# Autodesk Inventor assembly: RCS
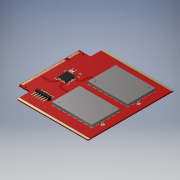
[picture p0: Inventor's stored thumbnail of the model, 180x180]
Saved by Autodesk Inventor 2018 (Build 220112000, 112)
## iProperties
Created: 2018-07-04
Part Number: RCS
Document SubType Name: Assembly
Designer: Bradley
Author: Bradley
## Documents named in this file (10)
- D:\Users\Bradley\Documents\CougsInSpace\CougSat1-Hardware\CougSat1-RadioBoard\CADModel\Native\Comms.iam
- D:\Users\Bradley\Documents\CougsInSpace\CougSat1-Hardware\CougSat1-RadioBoard\CADModel\Native\Comms_PCB.ipt
- D:\Users\Bradley\Documents\CougsInSpace\Resources\ComponentModels\Connectors\U.FL_Male.ipt
- D:\Users\Bradley\Documents\CougsInSpace\Resources\ComponentModels\Electronics\Crystal_ECX-42.ipt
- D:\Users\Bradley\Documents\CougsInSpace\Resources\ComponentModels\Electronics\LED_1608.ipt
- D:\Users\Bradley\Documents\CougsInSpace\Resources\ComponentModels\Connectors\SMD2.54-1x06-R.ipt
- D:\Users\Bradley\Documents\CougsInSpace\Resources\ComponentModels\Electronics\Shield_Frame-40x30mm.ipt
- D:\Users\Bradley\Documents\CougsInSpace\Resources\ComponentModels\Electronics\Shield_Cover-40x30mm.ipt
- D:\Users\Bradley\Documents\CougsInSpace\Resources\ComponentModels\Electronics\Capacitor_1608-0.8mm.ipt
- D:\Users\Bradley\Documents\CougsInSpace\Resources\ComponentModels\Electronics\Semiconductor_QFP64-10x10.ipt
## Components (17 placed, 9 different names)
1. Comms_PCB:1 — Mate:11, Mate:12, Mate:16, Mate:20, Flush:14, Mate:21, Mate:22, Flush:15, Mate:23, Flush:16, Flush:17, Mate:24, Flush:18, Flush:19, Mate:25, Mate:26, Mate:27, Mate:28, Mate:33, Flush:21, Flush:22, Mate:34, Mate:35, Mate:36, Mate:37, Flush:27, Mate:29, Mate:30, Mate:38, Mate:39, Flush:30, Flush:31, Mate:31, Mate:40, Flush:33, Mate:32, Mate:41, Flush:35
2. U.FL_Male:1 — Flush:11, Mate:2, Mate:11, Flush:12, Flush:13
3. Crystal_ECX-42:1 — Mate:24, Flush:18, Flush:19
4. LED_1608:1 — Mate:31, Mate:40, Flush:33
5. SMD2.54-1x06-R:1 — Mate:23, Flush:16, Flush:17
6. U.FL_Male:2 — Mate:12, Flush:12, Flush:13
7. Shield_Frame-40x30mm:1 — Mate:13, Mate:14, Mate:15, Mate:16, Flush:14, Mate:21
8. Shield_Cover-40x30mm:1 — Mate:13, Mate:14, Mate:15
9. Shield_Frame-40x30mm:2 — Mate:20, Mate:22, Flush:15
10. Shield_Cover-40x30mm:2
11. Capacitor_1608-0.8mm:1 — Mate:26, Flush:22, Mate:36
12. Capacitor_1608-0.8mm:2 — Mate:27, Flush:21, Mate:37
13. Capacitor_1608-0.8mm:3 — Mate:25, Mate:34, Mate:35
14. Capacitor_1608-0.8mm:4 — Mate:28, Mate:33, Flush:27
15. Capacitor_1608-0.8mm:5 — Mate:30, Mate:38, Flush:30
16. Capacitor_1608-0.8mm:6 — Mate:29, Mate:39, Flush:31
17. Semiconductor_QFP64-10x10:1 — Mate:32, Mate:41, Flush:35
## Relationships (48: Mate 32, Flush 16)
- Flush:11 (-15 mm): U.FL_Male:1
- Mate:2 (85 mm): U.FL_Male:1
- Mate:11: Comms_PCB:1 ↔ U.FL_Male:1
- Mate:12: Comms_PCB:1 ↔ U.FL_Male:2
- Flush:12: U.FL_Male:1 ↔ U.FL_Male:2
- Flush:13 (-40 mm): U.FL_Male:1 ↔ U.FL_Male:2
- Mate:13: Shield_Frame-40x30mm:1 ↔ Shield_Cover-40x30mm:1
- Mate:14 (0.1 mm): Shield_Frame-40x30mm:1 ↔ Shield_Cover-40x30mm:1
- Mate:15 (0.1 mm): Shield_Frame-40x30mm:1 ↔ Shield_Cover-40x30mm:1
- Mate:16: Comms_PCB:1 ↔ Shield_Frame-40x30mm:1
- [Mate]: Shield_Frame-40x30mm:2 ↔ Shield_Cover-40x30mm:2
- [Mate] (0.1 mm): Shield_Frame-40x30mm:2 ↔ Shield_Cover-40x30mm:2
- [Mate] (0.1 mm): Shield_Frame-40x30mm:2 ↔ Shield_Cover-40x30mm:2
- Mate:20: Comms_PCB:1 ↔ Shield_Frame-40x30mm:2
- Flush:14 (1.1 mm): Comms_PCB:1 ↔ Shield_Frame-40x30mm:1
- Mate:21 (-1.1 mm): Comms_PCB:1 ↔ Shield_Frame-40x30mm:1
- Mate:22 (-1.1 mm): Comms_PCB:1 ↔ Shield_Frame-40x30mm:2
- Flush:15 (1.1 mm): Comms_PCB:1 ↔ Shield_Frame-40x30mm:2
- Mate:23: Comms_PCB:1 ↔ SMD2.54-1x06-R:1
- Flush:16 (0.18 mm): Comms_PCB:1 ↔ SMD2.54-1x06-R:1
- Flush:17 (-0.25 mm): Comms_PCB:1 ↔ SMD2.54-1x06-R:1
- Mate:24: Comms_PCB:1 ↔ Crystal_ECX-42:1
- Flush:18 (0.125 mm): Comms_PCB:1 ↔ Crystal_ECX-42:1
- Flush:19 (0.2 mm): Comms_PCB:1 ↔ Crystal_ECX-42:1
- Mate:25: Comms_PCB:1 ↔ Capacitor_1608-0.8mm:3
- Mate:26: Comms_PCB:1 ↔ Capacitor_1608-0.8mm:1
- Mate:27: Comms_PCB:1 ↔ Capacitor_1608-0.8mm:2
- Mate:28: Comms_PCB:1 ↔ Capacitor_1608-0.8mm:4
- Mate:33 (0.125 mm): Comms_PCB:1 ↔ Capacitor_1608-0.8mm:4
- Flush:21 (0.125 mm): Comms_PCB:1 ↔ Capacitor_1608-0.8mm:2
- Flush:22 (0.125 mm): Comms_PCB:1 ↔ Capacitor_1608-0.8mm:1
- Mate:34 (0.125 mm): Comms_PCB:1 ↔ Capacitor_1608-0.8mm:3
- Mate:35 (0.64 mm): Comms_PCB:1 ↔ Capacitor_1608-0.8mm:3
- Mate:36 (0.64 mm): Comms_PCB:1 ↔ Capacitor_1608-0.8mm:1
- Mate:37 (0.64 mm): Comms_PCB:1 ↔ Capacitor_1608-0.8mm:2
- Flush:27 (0.64 mm): Comms_PCB:1 ↔ Capacitor_1608-0.8mm:4
- Mate:29: Comms_PCB:1 ↔ Capacitor_1608-0.8mm:6
- Mate:30: Comms_PCB:1 ↔ Capacitor_1608-0.8mm:5
- Mate:38 (0.64 mm): Comms_PCB:1 ↔ Capacitor_1608-0.8mm:5
- Mate:39 (0.64 mm): Comms_PCB:1 ↔ Capacitor_1608-0.8mm:6
- Flush:30 (0.125 mm): Comms_PCB:1 ↔ Capacitor_1608-0.8mm:5
- Flush:31 (0.125 mm): Comms_PCB:1 ↔ Capacitor_1608-0.8mm:6
- Mate:31: Comms_PCB:1 ↔ LED_1608:1
- Mate:40 (0.6095 mm): Comms_PCB:1 ↔ LED_1608:1
- Flush:33 (0.15 mm): Comms_PCB:1 ↔ LED_1608:1
- Mate:32: Comms_PCB:1 ↔ Semiconductor_QFP64-10x10:1
- Mate:41 (0.35 mm): Comms_PCB:1 ↔ Semiconductor_QFP64-10x10:1
- Flush:35 (-0.35 mm): Comms_PCB:1 ↔ Semiconductor_QFP64-10x10:1
## Named parameters: d26_d22 = 0 mm, d27_d23 = 0.1 mm, d28_d24 = 0.1 mm
